# Autodesk Inventor assembly: Assembly1
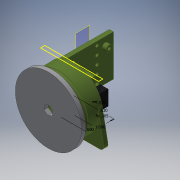
[picture p0: Inventor's stored thumbnail of the model, 180x180]
Saved by Autodesk Inventor 2018 (Build 220112000, 112)
## iProperties
Created: 2018-01-26
Part Number: Assembly1
Document SubType Name: Assembly
Designer: prakh
Author: prakh
## Documents named in this file (5)
- D:\GIT\ModernMobility\CADS\Alternate Wheel\Assembly1.iam
- D:\GIT\ModernMobility\CADS\Alternate Wheel\mounting plate.ipt
- D:\GIT\ModernMobility\CADS\Alternate Wheel\motor mount 2.ipt
- D:\GIT\ModernMobility\CADS\Alternate Wheel\Imported Components\microServo-sg90\microServo-sg90.ipt
- D:\GIT\ModernMobility\CADS\Alternate Wheel\wheel hub.ipt
## Components (4 placed, 4 different names)
1. mounting plate:1 — Mate:1, Mate:2, Mate:3, Mate:4, Mate:7, Mate:8, Mate:9
2. motor mount 2:1 — Mate:1, Mate:2, Mate:3
3. microServo-sg90:1 — Mate:4, Mate:8
4. wheel hub:1 — Mate:7, Mate:9
## Relationships (7: Mate 7)
- Mate:1: mounting plate:1 ↔ motor mount 2:1
- Mate:2: mounting plate:1 ↔ motor mount 2:1
- Mate:3: mounting plate:1 ↔ motor mount 2:1
- Mate:4: mounting plate:1 ↔ microServo-sg90:1
- Mate:7: mounting plate:1 ↔ wheel hub:1
- Mate:8: mounting plate:1 ↔ microServo-sg90:1
- Mate:9 (0.508 mm): mounting plate:1 ↔ wheel hub:1
